# Autodesk Inventor assembly: 01 ASY GBK wall shield 1.1.1
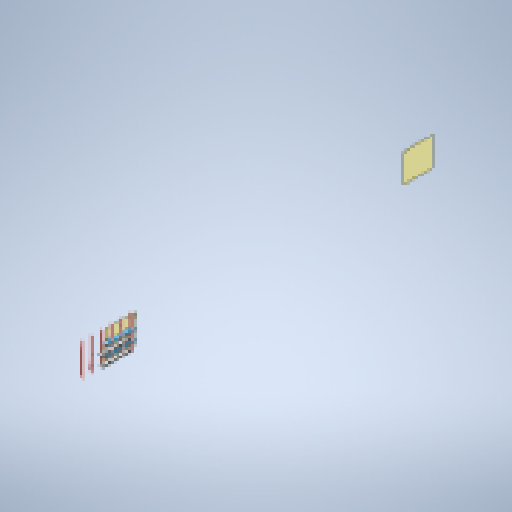
[picture p0: Inventor's stored thumbnail of the model, 512x512]
Saved by Autodesk Inventor 2026.2 (Build 302298000, 298)
## iProperties
Created: 2026-05-07
Part Number: 01 ASY GBK wall shield 1.1.1
Document SubType Name: Assembly
Designer: admin
Mass: 245734 g
Surface Area: 167509 cm^2
Volume: 31303.7 cm^3
Density: 7.85 g/cm^3
Author: admin
## Documents named in this file (5)
- C:\Users\admin\Documents\Inventor\GBK-Gubkinskiy\01 ASY GBK wall shield 1.1.1.iam
- C:\Users\admin\Documents\Inventor\GBK-Gubkinskiy\01.1 GBK shield.ipt
- C:\Users\admin\Documents\Inventor\GBK-Gubkinskiy\01.3 GBK stringer 1.ipt
- C:\Users\admin\Documents\Inventor\GBK-Gubkinskiy\0232 GBK stringer 2.ipt
- C:\Users\admin\Documents\Inventor\GBK-Gubkinskiy\01.2 GBK main rib.ipt
## Components (52 placed, 6 different names)
1. 0232 GBK stringer 2:1
2. 01.3 GBK stringer 1.ipt:1
3. 0232 GBK stringer 2:2
4. 0232 GBK stringer 2:3
5. 01.2 GBK main rib.ipt:1
6. 01.2 GBK main rib:2
7. 01.2 GBK main rib:3
8. 01.2 GBK main rib:4
9. 01.2 GBK main rib:5
10. 01.2 GBK main rib:6
11. 01.2 GBK main rib:7
12. 01.2 GBK main rib:8
13. 01.2 GBK main rib:9
14. 01.2 GBK main rib:10
15. 01.2 GBK main rib:11
16. 01.2 GBK main rib:12
17. 01.2 GBK main rib:13
18. 01.2 GBK main rib:14
19. 01.2 GBK main rib:15
20. 01.2 GBK main rib:16
21. 01.2 GBK main rib:17
22. 01.2 GBK main rib:18
23. 01.2 GBK main rib:19
24. 01.2 GBK main rib:20
25. 01.2 GBK main rib:21
26. 01.2 GBK main rib:22
27. 01.2 GBK main rib:23
28. 01.2 GBK main rib:24
29. 01.2 GBK main rib:25
30. 01.2 GBK main rib:26
31. 01.2 GBK main rib:27
32. 01.2 GBK main rib:28
33. 01.2 GBK main rib:29
34. 01.2 GBK main rib:30
35. 01.2 GBK main rib:31
36. 01.2 GBK main rib:32
37. 01.2 GBK main rib:33
38. 01.2 GBK main rib:34
39. 01.2 GBK main rib:35
40. 01.2 GBK main rib:36
41. 01.1 GBK shield.ipt:1
42. Part111:2
43. Part111:3
44. Part111:4
45. Part111:5
46. Part111:6
47. Part111:7
48. Part111:8
49. Part111:9
50. Part111:10
51. Part111:11
52. Part111:12
## Component patterns: (36 elements, first: 01.2 GBK main rib.ipt:1), (12 elements, first: 01.1 GBK shield.ipt:1)
## Relationships (5: Mate 2, WeldJoint 2, Flush 1)
- [Mate]: 01.2 GBK main rib.ipt:1 ↔ 01.1 GBK shield.ipt:1
- [Flush] (250 mm): 01.2 GBK main rib.ipt:1 ↔ 01.1 GBK shield.ipt:1
- [Mate]: 01.2 GBK main rib.ipt:1 ↔ 01.1 GBK shield.ipt:1
- [WeldJoint] (4 mm): 01.3 GBK stringer 1.ipt:1 ↔ 01.2 GBK main rib.ipt:1
- [WeldJoint] (4 mm): 0232 GBK stringer 2:1 ↔ 01.2 GBK main rib.ipt:1
